# Autodesk Inventor assembly: enclosure_asus.ipt
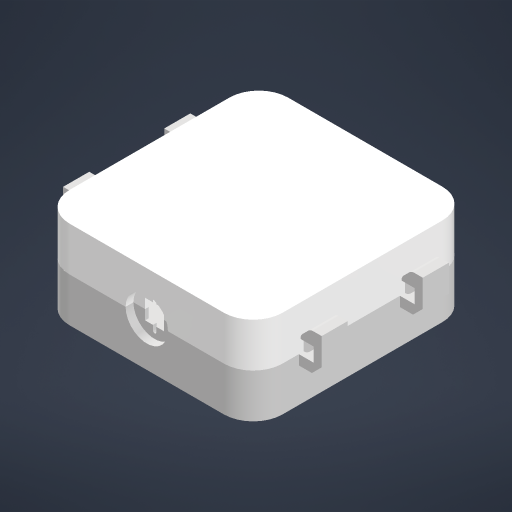
[picture p0: Inventor's stored thumbnail of the model, 512x512]
Saved by Autodesk Inventor 2024 (Build 280153000, 153)
## iProperties
Created: 2023-07-19
Part Number: enclosure_asus.ipt
Document SubType Name: Assembly
Designer: LabTel_Admin
Author: LabTel_Admin
## Documents named in this file (3)
- C:\Users\luisf\OneDrive - ESCUELA COLOMBIANA DE INGENIERIA JULIO GARAVITO\Documents\Inventor\Projects\enclosure_asus\enclosure_asus_asembly.ipt.iam
- C:\Users\luisf\OneDrive - ESCUELA COLOMBIANA DE INGENIERIA JULIO GARAVITO\Documents\Inventor\Projects\enclosure_asus\enclosure_down.ipt
- C:\Users\luisf\OneDrive - ESCUELA COLOMBIANA DE INGENIERIA JULIO GARAVITO\Documents\Inventor\Projects\enclosure_asus\enclosure_up.ipt
## Components (2 placed, 2 different names)
1. enclosure_down:1 — Coincidencia:2, Nivelación:3, Nivelación:4, Nivelación:5
2. enclosure_up:1 — Coincidencia:2, Nivelación:3, Nivelación:4, Nivelación:5
## Relationships (4: Flush 3, Mate 1)
- Coincidencia:2 [Mate]: enclosure_down:1 ↔ enclosure_up:1
- Nivelación:3 [Flush]: enclosure_down:1 ↔ enclosure_up:1
- Nivelación:4 [Flush]: enclosure_down:1 ↔ enclosure_up:1
- Nivelación:5 [Flush]: enclosure_down:1 ↔ enclosure_up:1
